# Autodesk Inventor assembly: Assembly1
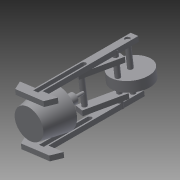
[picture p0: Inventor's stored thumbnail of the model, 180x180]
Saved by Autodesk Inventor 2015 (Build 190159000, 159)
## iProperties
Created: 2014-07-15
Part Number: Assembly1
Document SubType Name: Assembly
Designer: shohei
Author: shohei
## Documents named in this file (9)
- C:\Users\shohei\Documents\Inventor\FufuPounder\Assembly1.iam
- C:\Users\shohei\Documents\Inventor\FufuPounder\mortar.ipt
- C:\Users\shohei\Documents\Inventor\FufuPounder\Part1.ipt
- C:\Users\shohei\Documents\Inventor\FufuPounder\mallet.ipt
- C:\Users\shohei\Documents\Inventor\FufuPounder\shaft.ipt
- C:\Users\shohei\Documents\Inventor\FufuPounder\Part2.ipt
- C:\Users\shohei\Documents\Inventor\FufuPounder\pulley.ipt
- C:\Users\shohei\Documents\Inventor\FufuPounder\Part4.ipt
- C:\Users\shohei\Documents\Inventor\FufuPounder\Part5.ipt
## Components (11 placed, 8 different names)
1. mortar:1 — Flush:1, Flush:2, Cylindrical:1, Mate:1
2. Part1:1 — Flush:1, Flush:3, Rigid:2
3. Part1:2 — Flush:2, Flush:3
4. mallet:1 — Rigid:1
5. shaft:1 — Rigid:1, Cylindrical:1
6. pulley:1 — Cylindrical:7, Cylindrical:11
7. Part2:2 — Cylindrical:5, Cylindrical:6, Cylindrical:7
8. Part4:1 — Cylindrical:5, Cylindrical:9
9. Part4:2 — Cylindrical:6, Cylindrical:10
10. Part2:3 — Rigid:2, Cylindrical:11
11. Part5:1 — Cylindrical:9, Cylindrical:10
## Relationships (13: CylindricalJoint 7, Flush 3, WeldJoint 2, Mate 1)
- Flush:1: mortar:1 ↔ Part1:1
- Flush:2: mortar:1 ↔ Part1:2
- Rigid:1 [WeldJoint]: mallet:1 ↔ shaft:1
- Cylindrical:1: mortar:1 ↔ shaft:1
- Cylindrical:5: Part2:2 ↔ Part4:1
- Cylindrical:6: Part2:2 ↔ Part4:2
- Cylindrical:7: pulley:1 ↔ Part2:2
- Mate:1: mortar:1
- Flush:3: Part1:1 ↔ Part1:2
- Rigid:2 [WeldJoint]: Part1:1 ↔ Part2:3
- Cylindrical:9: Part4:1 ↔ Part5:1
- Cylindrical:10: Part4:2 ↔ Part5:1
- Cylindrical:11: pulley:1 ↔ Part2:3
